# Autodesk Inventor assembly: Assembly2
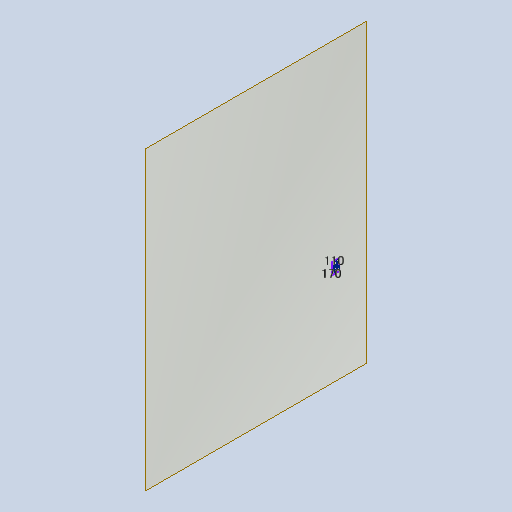
[picture p0: Inventor's stored thumbnail of the model, 512x512]
Saved by Autodesk Inventor 2025.1 (Build 291241000, 241)
## iProperties
Created: 2024-12-09
Part Number: Assembly2
Document SubType Name: Assembly
Designer: haruy
Author: haruy
## Documents named in this file (5)
- C:\Users\haruy\Documents\ロボコン\NHK2025\cad\cnc\Assembly2.iam
- C:\Users\haruy\Documents\ロボコン\NHK2025\cad\nagahisa\dribl\R2-Rzvector\RZvector-v1-MP-Tr-F.ipt
- C:\Users\haruy\Documents\ロボコン\NHK2025\cad\nagahisa\dribl\R2-Rzvector\RZvector-v1-Plate-P-TB-F.ipt
- C:\Users\haruy\Documents\ロボコン\NHK2025\cad\nagahisa\base_weel\base_weel-v1-Plate-expand-1.ipt
- C:\Users\haruy\Documents\ロボコン\NHK2025\cad\nagahisa\base_weel\base_weel-v1-Plate-expand-2.ipt
## Components (8 placed, 4 different names)
1. RZvector-v1-MP-Tr-F:1 — フラッシュ:1, メイト:3
2. RZvector-v1-MP-Tr-F:2 — フラッシュ:2, メイト:2, フラッシュ:10
3. RZvector-v1-Plate-P-TB-F:1 — フラッシュ:3
4. RZvector-v1-Plate-P-TB-F:2 — フラッシュ:4, メイト:6, フラッシュ:13
5. base_weel-v1-Plate-expand-1:1 — フラッシュ:6, フラッシュ:9, メイト:1, メイト:2, フラッシュ:10
6. base_weel-v1-Plate-expand-1:2 — フラッシュ:5, フラッシュ:9, メイト:1, メイト:3, メイト:6, フラッシュ:13
7. base_weel-v1-Plate-expand-2:1 — フラッシュ:8, フラッシュ:12, メイト:5
8. base_weel-v1-Plate-expand-2:2 — フラッシュ:7, フラッシュ:12, メイト:5
## Relationships (17: Flush 12, Mate 5)
- フラッシュ:1 [Flush]: RZvector-v1-MP-Tr-F:1
- フラッシュ:2 [Flush]: RZvector-v1-MP-Tr-F:2
- フラッシュ:3 [Flush]: RZvector-v1-Plate-P-TB-F:1
- フラッシュ:4 [Flush]: RZvector-v1-Plate-P-TB-F:2
- フラッシュ:5 [Flush]: base_weel-v1-Plate-expand-1:2
- フラッシュ:6 [Flush]: base_weel-v1-Plate-expand-1:1
- フラッシュ:7 [Flush]: base_weel-v1-Plate-expand-2:2
- フラッシュ:8 [Flush]: base_weel-v1-Plate-expand-2:1
- フラッシュ:9 [Flush]: base_weel-v1-Plate-expand-1:1 ↔ base_weel-v1-Plate-expand-1:2
- メイト:1 [Mate] (5 mm): base_weel-v1-Plate-expand-1:1 ↔ base_weel-v1-Plate-expand-1:2
- メイト:2 [Mate] (5 mm): RZvector-v1-MP-Tr-F:2 ↔ base_weel-v1-Plate-expand-1:1
- フラッシュ:10 [Flush]: RZvector-v1-MP-Tr-F:2 ↔ base_weel-v1-Plate-expand-1:1
- メイト:3 [Mate] (5 mm): RZvector-v1-MP-Tr-F:1 ↔ base_weel-v1-Plate-expand-1:2
- フラッシュ:12 [Flush]: base_weel-v1-Plate-expand-2:1 ↔ base_weel-v1-Plate-expand-2:2
- メイト:5 [Mate] (5 mm): base_weel-v1-Plate-expand-2:1 ↔ base_weel-v1-Plate-expand-2:2
- メイト:6 [Mate] (5 mm): RZvector-v1-Plate-P-TB-F:2 ↔ base_weel-v1-Plate-expand-1:2
- フラッシュ:13 [Flush]: RZvector-v1-Plate-P-TB-F:2 ↔ base_weel-v1-Plate-expand-1:2
